# Autodesk Inventor assembly: HbFinger01ForChild_MIR1
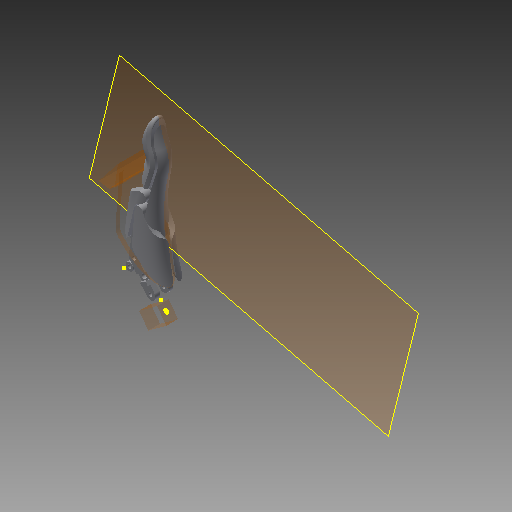
[picture p0: Inventor's stored thumbnail of the model, 512x512]
Saved by Autodesk Inventor 2017.3 (Build 213256000, 256)
## iProperties
Part Number: HbFinger01ForChild_MIR1
Material: 一般
Document SubType Name: Assembly
Designer: sktom
Author: sktom
## Documents named in this file (7)
- D:\CloudStrage\OneDrive\CAD\MAJ\hackberry\HACKberry-hardware\3D_69%inlength\Inventor\HbHandForChild\HbFinger01ForChild\HbFinger01ForChild_MIR1.iam
- D:\CloudStrage\OneDrive\CAD\MAJ\hackberry\HACKberry-hardware\3D_69%inlength\Inventor\HbHandForChild\HbFinger01ForChild\HbCouplerLinkCover03ForChild_MIR1.ipt
- D:\CloudStrage\OneDrive\CAD\MAJ\hackberry\HACKberry-hardware\3D_69%inlength\Inventor\HbHandForChild\HbFinger01ForChild\HbCouplerLink02ForChild_MIR1.ipt
- D:\CloudStrage\OneDrive\CAD\MAJ\hackberry\HACKberry-hardware\3D_69%inlength\Inventor\HbHandForChild\HbFinger01ForChild\HbMiddle-DistalPhalanx02ForChild_MIR1.ipt
- D:\CloudStrage\OneDrive\CAD\MAJ\hackberry\HACKberry-hardware\3D_69%inlength\Inventor\HbHandForChild\HbFinger01ForChild\HbProximalPhalanx02ForChild_MIR1.ipt
- D:\CloudStrage\OneDrive\CAD\MAJ\hackberry\HACKberry-hardware\3D_69%inlength\Inventor\HbHandForChild\HbFinger01ForChild\HbProximalPhalanxCover02ForChild_MIR1.ipt
- D:\CloudStrage\OneDrive\CAD\MAJ\hackberry\HACKberry-hardware\3D_69%inlength\Inventor\HbHandForChild\HbFinger01ForChild\shaft_phi1.5_l6_MIR.ipt
## Components (7 placed, 6 different names)
1. HbCouplerLinkCover03ForChild_MIR1:1 — 挿入:2, 挿入:1
2. HbCouplerLink02ForChild_MIR1:1 — 挿入:2, 挿入:1, 挿入:3, 挿入:8
3. HbMiddle-DistalPhalanx02ForChild_MIR1:1 — 挿入:3, 挿入:4, 円柱状:2
4. HbProximalPhalanx02ForChild_MIR1:1 — 挿入:6, 挿入:5
5. HbProximalPhalanxCover02ForChild_MIR1:1 — 挿入:6, 挿入:5, 挿入:4, 挿入:7
6. shaft_phi1.5_l6_MIR:1 — 挿入:7
7. shaft_phi1.5_l6_MIR:2 — 挿入:8, 円柱状:2
## Relationships (9: Insert 8, CylindricalJoint 1)
- 挿入:2 [Insert]: HbCouplerLinkCover03ForChild_MIR1:1 ↔ HbCouplerLink02ForChild_MIR1:1
- 挿入:1 [Insert]: HbCouplerLinkCover03ForChild_MIR1:1 ↔ HbCouplerLink02ForChild_MIR1:1
- 挿入:3 [Insert] (0.4 mm): HbCouplerLink02ForChild_MIR1:1 ↔ HbMiddle-DistalPhalanx02ForChild_MIR1:1
- 挿入:6 [Insert]: HbProximalPhalanx02ForChild_MIR1:1 ↔ HbProximalPhalanxCover02ForChild_MIR1:1
- 挿入:5 [Insert]: HbProximalPhalanx02ForChild_MIR1:1 ↔ HbProximalPhalanxCover02ForChild_MIR1:1
- 挿入:4 [Insert] (0.4 mm): HbMiddle-DistalPhalanx02ForChild_MIR1:1 ↔ HbProximalPhalanxCover02ForChild_MIR1:1
- 挿入:7 [Insert] (0.5 mm): HbProximalPhalanxCover02ForChild_MIR1:1 ↔ shaft_phi1.5_l6_MIR:1
- 挿入:8 [Insert] (0.5 mm): HbCouplerLink02ForChild_MIR1:1 ↔ shaft_phi1.5_l6_MIR:2
- 円柱状:2 [CylindricalJoint]: HbMiddle-DistalPhalanx02ForChild_MIR1:1 ↔ shaft_phi1.5_l6_MIR:2
